# Autodesk Inventor assembly: esc
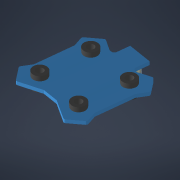
[picture p0: Inventor's stored thumbnail of the model, 180x180]
Saved by Autodesk Inventor 2022 (Build 260153000, 153)
## iProperties
Created: 2022-07-21
Part Number: esc
Document SubType Name: Assembly
Designer: ancher
Author: ancher
## Documents named in this file (3)
- E:\RC\print_3d\aos5\esc.iam
- E:\RC\print_3d\aos5\esc.ipt
- E:\RC\print_3d\aos5\rubber_sleeve.ipt
## Components (5 placed, 2 different names)
1. esc:1 — Mate:1, Mate:2, Mate:3, Mate:4, Mate:5, Mate:6, Mate:7, Mate:8
2. rubber_sleeve:1 — Mate:3, Mate:7
3. rubber_sleeve:2 — Mate:4, Mate:5
4. rubber_sleeve:3 — Mate:1, Mate:6
5. rubber_sleeve:4 — Mate:2, Mate:8
## Relationships (8: Mate 8)
- Mate:1: esc:1 ↔ rubber_sleeve:3
- Mate:2: esc:1 ↔ rubber_sleeve:4
- Mate:3: esc:1 ↔ rubber_sleeve:1
- Mate:4: esc:1 ↔ rubber_sleeve:2
- Mate:5: esc:1 ↔ rubber_sleeve:2
- Mate:6: esc:1 ↔ rubber_sleeve:3
- Mate:7: esc:1 ↔ rubber_sleeve:1
- Mate:8: esc:1 ↔ rubber_sleeve:4
